# Autodesk Inventor assembly: KN-00-03-00
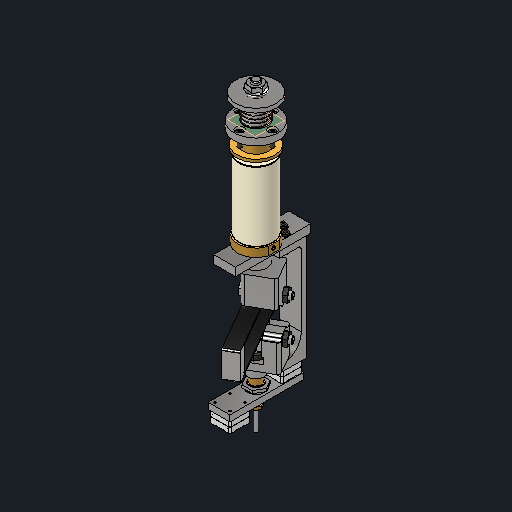
[picture p0: Inventor's stored thumbnail of the model, 512x512]
Saved by Autodesk Inventor 2025.2 (Build 292293000, 293)
## iProperties
Created: 2025-03-24
Part Number: KN-00-03-00
Document SubType Name: Assembly
Designer: Kacper Mik
Mass: 1101.42 g
Surface Area: 706.876 cm^2
Volume: 148.025 cm^3
Density: 7.44076 g/cm^3
Author: Kacper Mik
## Documents named in this file (32)
- C:\Users\kacpe\Documents\STUDIA\INŻYNIERKA\Nanotwardościomierz\Nanotwardosciomierz inventor\03-00-zesp_referencji.iam
- 03-00-zesp_wgłębnika.iam
- C:\Users\kacpe\Documents\STUDIA\INŻYNIERKA\Nanotwardościomierz\Nanotwardosciomierz inventor\Pobrane\Uchwyt do wgłębnika.ipt
- C:\Users\kacpe\Documents\STUDIA\INŻYNIERKA\Nanotwardościomierz\Nanotwardosciomierz inventor\02-01-ind_plytkaC1.ipt
- C:\Users\kacpe\Documents\STUDIA\INŻYNIERKA\Nanotwardościomierz\Nanotwardosciomierz inventor\02-01-ind_tulejaC1.ipt
- C:\Users\kacpe\Documents\STUDIA\INŻYNIERKA\Nanotwardościomierz\Nanotwardosciomierz inventor\02-01-dociskC1.ipt
- C:\Users\kacpe\Documents\STUDIA\INŻYNIERKA\Nanotwardościomierz\Nanotwardosciomierz inventor\02-04-ind_trzpien.ipt
- C:\Users\kacpe\Documents\STUDIA\INŻYNIERKA\Nanotwardościomierz\Nanotwardosciomierz inventor\P-025.40H Piezo Ring Actuators.ipt
- C:\Users\kacpe\Documents\STUDIA\INŻYNIERKA\Nanotwardościomierz\Nanotwardosciomierz inventor\Łożysko liniowe z kołnierzem okrągłym LMF08UU-L.ipt
- C:\Users\kacpe\Documents\STUDIA\INŻYNIERKA\Nanotwardościomierz\Nanotwardosciomierz inventor\02-06-tuleja_A0.ipt
- C:\Users\kacpe\Documents\STUDIA\INŻYNIERKA\Nanotwardościomierz\Nanotwardosciomierz inventor\CC\en-US\ISO 7045  H\ISO 7045 - M3 x 8_ - 4.8 - H - ISO.ipt
- C:\Users\kacpe\Documents\STUDIA\INŻYNIERKA\Nanotwardościomierz\Nanotwardosciomierz inventor\zesp_czujnikow.iam
- C:\Users\kacpe\Documents\STUDIA\INŻYNIERKA\Nanotwardościomierz\Nanotwardosciomierz inventor\02-07-zawieszka_K1\02-07-zawieszka_K1.ipt
- C:\Users\kacpe\Documents\STUDIA\INŻYNIERKA\Nanotwardościomierz\Nanotwardosciomierz inventor\CC\en-US\ISO 4036(2)\ISO 4036 - M6(2).ipt
- C:\Users\kacpe\Documents\STUDIA\INŻYNIERKA\Nanotwardościomierz\Nanotwardosciomierz inventor\CC\en-US\ISO 4036(2)\ISO 4036 - M5(2).ipt
- C:\Users\kacpe\Documents\STUDIA\INŻYNIERKA\Nanotwardościomierz\Nanotwardosciomierz inventor\Zawias.ipt
- C:\Users\kacpe\Documents\STUDIA\INŻYNIERKA\Nanotwardościomierz\Nanotwardosciomierz inventor\CC\en-US\ISO 4014(2)\ISO 4014 - M5 x 25 - ISO.ipt
- C:\Users\kacpe\Documents\STUDIA\INŻYNIERKA\Nanotwardościomierz\Nanotwardosciomierz inventor\02-08-ind_trzpien_gora.ipt
- C:\Users\kacpe\Documents\STUDIA\INŻYNIERKA\Nanotwardościomierz\Nanotwardosciomierz inventor\02-09-plyta_C1.ipt
- C:\Users\kacpe\Documents\STUDIA\INŻYNIERKA\Nanotwardościomierz\Nanotwardosciomierz inventor\02-11-plyta_dolnaA1.ipt
- C:\Users\kacpe\Documents\STUDIA\INŻYNIERKA\Nanotwardościomierz\Nanotwardosciomierz inventor\02-12-tuleja_dolnaA1.ipt
- C:\Users\kacpe\Documents\STUDIA\INŻYNIERKA\Nanotwardościomierz\Nanotwardosciomierz inventor\CC\en-US\ISO 7089\ISO 7089 - 2 - 140 HV(1).ipt
- C:\Users\kacpe\Documents\STUDIA\INŻYNIERKA\Nanotwardościomierz\Nanotwardosciomierz inventor\CC\en-US\ISO 7045  H\ISO 7045 - M2 x 14_ - 4.8 - H - ISO.ipt
- C:\Users\kacpe\Documents\STUDIA\INŻYNIERKA\Nanotwardościomierz\Nanotwardosciomierz inventor\CC\en-US\ISO 4036(2)\ISO 4036 - M2(2).ipt
- C:\Users\kacpe\Documents\STUDIA\INŻYNIERKA\Nanotwardościomierz\Nanotwardosciomierz inventor\CC\en-US\ISO 7045  H\ISO 7045 - M2 x 8_ - 4.8 - H - ISO.ipt
- C:\Users\kacpe\Documents\STUDIA\INŻYNIERKA\Nanotwardościomierz\Nanotwardosciomierz inventor\CC\en-US\ISO 4766(2)\ISO 4766 - M3 x 8 - ISO.ipt
- C:\Users\kacpe\Documents\STUDIA\INŻYNIERKA\Nanotwardościomierz\Nanotwardosciomierz inventor\02-14-podkladka_K3.ipt
- C:\Users\kacpe\Documents\STUDIA\INŻYNIERKA\Nanotwardościomierz\Nanotwardosciomierz inventor\CC\en-US\ISO 4161\ISO 4161 - M6(1).ipt
- C:\Users\kacpe\Documents\STUDIA\INŻYNIERKA\Nanotwardościomierz\Nanotwardosciomierz inventor\02-15-sprezyna_K3.ipt
- C:\Users\kacpe\Documents\STUDIA\INŻYNIERKA\Nanotwardościomierz\Nanotwardosciomierz inventor\02-15-prowadzenie_K3.ipt
- C:\Users\kacpe\Documents\STUDIA\INŻYNIERKA\Nanotwardościomierz\Nanotwardosciomierz inventor\03-01-glowica_referencyjna.ipt
- C:\Users\kacpe\Documents\STUDIA\INŻYNIERKA\Nanotwardościomierz\Nanotwardosciomierz inventor\CC\en-US\CNS 4355\CNS 4355 - M 1,4 x 6.ipt
## Components (59 placed, 30 different names)
1. 03-01-glowica_referencyjna:1
2. CNS 4355 M 1,4 x 6:5 — Insert:65
3. CNS 4355 M 1,4 x 6:6 — Insert:64
4. CNS 4355 M 1,4 x 6:7 — Insert:63
5. CNS 4355 M 1,4 x 6:8 — Insert:62
6. zesp_czujnikow:3 [sub-assembly] — Insert:66, Insert:67, Insert:68, Insert:69, Insert:70, Insert:71
7. CNS 4355 M 1,4 x 6:9 — Insert:71
8. CNS 4355 M 1,4 x 6:10 — Insert:70
9. CNS 4355 M 1,4 x 6:11 — Insert:69
10. CNS 4355 M 1,4 x 6:12 — Insert:68
11. 02-14-podkladka_K3:1 — Insert:45, Insert:46
12. 02-15-prowadzenie_K3:1 — Insert:55
13. 02-15-sprezyna_K3:1 — Mate:20, Mate:21
14. 02-01-ind_plytkaC1:1 — Angle:1, Insert:2, Insert:7, Insert:15, Insert:16, Insert:66, Insert:67
15. 02-02-ind_tulejaC1:1 — Insert:2, Insert:5, Insert:6
16. 02-03-docisk:1 — Insert:7, Angle:2
17. 02-04-ind_trzpien_dolny:1 — Insert:6, Insert:19
18. 02-06-tuleja_A0:1 — Insert:12, Insert:56
19. 02-07-zawieszka_K1:1 — Angle:4, Insert:21, Angle:5, Insert:22, Angle:6, Insert:24, Insert:25
20. 02-08-zawias — Insert:19, Insert:20, Insert:21, Angle:5, Insert:23
21. 02-08-zawias:2 — Angle:6, Insert:24, Insert:26, Insert:27, Insert:28
22. 02-09-plyta_C1:1 — Insert:29, Insert:30, Insert:32, Insert:51, Insert:52
23. 02-10-ind_trzpien_gora:1 — Insert:27, Insert:31, Insert:45
24. 02-11-plyta_dolnaA1:1 — Insert:31, Angle:7, Insert:36, Insert:40, Insert:53, Insert:54, Angle:8
25. 02-12-tuleja_dolnaA1:1 — Insert:40, Insert:41, Insert:42, Insert:43, Insert:44, Angle:8
26. CNS 4355 M 1,4 x 6:4 — Insert:59
27. CNS 4355 M 1,4 x 6:2 — Insert:60
28. CNS 4355 M 1,4 x 6:3 — Insert:58
29. CNS 4355 M 1,4 x 6:1 — Insert:61
30. ISO 7089 2:7 — Insert:53
31. ISO 7089 2:6 — Insert:52
32. ISO 4036 M2:3
33. ISO 7089 2:5 — Insert:54
34. ISO 7045 H M2 x 14 - 4.8 - H:3
35. ISO 4036 M2:2
36. ISO 7089 2:4 — Insert:51
37. ISO 7045 H M2 x 14 - 4.8 - H:2
38. ISO 4161 M6:1 — Insert:46
39. ISO 4766 M3 x 8:1 — Insert:43
40. ISO 7045 H M2 x 8 - 4.8 - H:2 — Insert:42
41. ISO 7045 H M2 x 8 - 4.8 - H:1 — Insert:41
42. ISO 7089 2:3 — Insert:36, Insert:37
43. ISO 4036 M2:1 — Insert:37
44. ISO 7089 2:1 — Insert:32, Insert:33
45. ISO 7045 H M2 x 14 - 4.8 - H:1 — Insert:33
46. ISO 4014 M5 x 25:2 — Insert:25
47. ISO 4036 M5:2 — Insert:26
48. ISO 4036 M6:2 — Insert:28
49. ISO 4036 M5:1 — Insert:23
50. ISO 4036 M6:1 — Insert:20
51. ISO 4014 M5 x 25:1 — Insert:22
52. ISO 7045 H M3 x 8 - 4.8 - H:4 — Mate:8
53. ISO 7045 H M3 x 8 - 4.8 - H:3 — Mate:6
54. ISO 7045 H M3 x 8 - 4.8 - H:2 — Mate:4
55. ISO 7045 H M3 x 8 - 4.8 - H:1 — Mate:2
56. P-025.40H Piezo Ring Actuators:1 — Insert:12, Insert:44
57. LMF08UU-L-Łożysko liniowe z kołnierzem okrągłym:1 — Angle:3, Mate:2, Mate:4, Mate:6, Mate:8, Mate:19, Mate:21, Insert:55, Insert:56
58. Uchwyt do wgłębnika:1 — Insert:5, Angle:2
59. zesp_czujnikow:2 [sub-assembly] — Insert:15, Insert:16, Insert:29, Insert:30, Insert:58, Insert:59, Insert:60, Insert:61, Insert:62, Insert:63, Insert:64, Insert:65
## Relationships (70: Insert 55, Angle 8, Mate 7)
- Angle:1 (0 deg): 02-01-ind_plytkaC1:1
- Insert:2: 02-01-ind_plytkaC1:1 ↔ 02-02-ind_tulejaC1:1
- Insert:5: 02-02-ind_tulejaC1:1 ↔ Uchwyt do wgłębnika:1
- Insert:6: 02-02-ind_tulejaC1:1 ↔ 02-04-ind_trzpien_dolny:1
- Insert:7: 02-01-ind_plytkaC1:1 ↔ 02-03-docisk:1
- Angle:2 (0 deg): 02-03-docisk:1 ↔ Uchwyt do wgłębnika:1
- Angle:3 (0 deg): LMF08UU-L-Łożysko liniowe z kołnierzem okrągłym:1
- Mate:2: ISO 7045 H M3 x 8 - 4.8 - H:1 ↔ LMF08UU-L-Łożysko liniowe z kołnierzem okrągłym:1
- Mate:4: ISO 7045 H M3 x 8 - 4.8 - H:2 ↔ LMF08UU-L-Łożysko liniowe z kołnierzem okrągłym:1
- Mate:6: ISO 7045 H M3 x 8 - 4.8 - H:3 ↔ LMF08UU-L-Łożysko liniowe z kołnierzem okrągłym:1
- Mate:8: ISO 7045 H M3 x 8 - 4.8 - H:4 ↔ LMF08UU-L-Łożysko liniowe z kołnierzem okrągłym:1
- Insert:12 (-0.2 mm): 02-06-tuleja_A0:1 ↔ P-025.40H Piezo Ring Actuators:1
- Insert:15: 02-01-ind_plytkaC1:1 ↔ zesp_czujnikow:2
- Insert:16: 02-01-ind_plytkaC1:1 ↔ zesp_czujnikow:2
- Angle:4 (60 deg): 02-07-zawieszka_K1:1
- Insert:19: 02-04-ind_trzpien_dolny:1 ↔ 02-08-zawias
- Insert:20: 02-08-zawias ↔ ISO 4036 M6:1
- Insert:21: 02-07-zawieszka_K1:1 ↔ 02-08-zawias
- Angle:5 (0 deg): 02-07-zawieszka_K1:1 ↔ 02-08-zawias
- Insert:22: 02-07-zawieszka_K1:1 ↔ ISO 4014 M5 x 25:1
- Insert:23: 02-08-zawias ↔ ISO 4036 M5:1
- Angle:6 (180 deg): 02-07-zawieszka_K1:1 ↔ 02-08-zawias:2
- Insert:24: 02-07-zawieszka_K1:1 ↔ 02-08-zawias:2
- Insert:25: 02-07-zawieszka_K1:1 ↔ ISO 4014 M5 x 25:2
- Insert:26: 02-08-zawias:2 ↔ ISO 4036 M5:2
- Insert:27: 02-08-zawias:2 ↔ 02-10-ind_trzpien_gora:1
- Insert:28: 02-08-zawias:2 ↔ ISO 4036 M6:2
- Insert:29: 02-09-plyta_C1:1 ↔ zesp_czujnikow:2
- Insert:30: 02-09-plyta_C1:1 ↔ zesp_czujnikow:2
- Insert:31: 02-10-ind_trzpien_gora:1 ↔ 02-11-plyta_dolnaA1:1
- Angle:7 (0 deg): 02-11-plyta_dolnaA1:1
- Insert:32: 02-09-plyta_C1:1 ↔ ISO 7089 2:1
- Insert:33: ISO 7089 2:1 ↔ ISO 7045 H M2 x 14 - 4.8 - H:1
- Insert:36: 02-11-plyta_dolnaA1:1 ↔ ISO 7089 2:3
- Insert:37: ISO 7089 2:3 ↔ ISO 4036 M2:1
- Mate:19: LMF08UU-L-Łożysko liniowe z kołnierzem okrągłym:1
- Insert:40: 02-11-plyta_dolnaA1:1 ↔ 02-12-tuleja_dolnaA1:1
- Insert:41: 02-12-tuleja_dolnaA1:1 ↔ ISO 7045 H M2 x 8 - 4.8 - H:1
- Insert:42: 02-12-tuleja_dolnaA1:1 ↔ ISO 7045 H M2 x 8 - 4.8 - H:2
- Insert:43 (0.35 mm): 02-12-tuleja_dolnaA1:1 ↔ ISO 4766 M3 x 8:1
- Insert:44: 02-12-tuleja_dolnaA1:1 ↔ P-025.40H Piezo Ring Actuators:1
- Insert:45: 02-14-podkladka_K3:1 ↔ 02-10-ind_trzpien_gora:1
- Insert:46: 02-14-podkladka_K3:1 ↔ ISO 4161 M6:1
- [Insert]: ISO 7089 2:4 ↔ ISO 7045 H M2 x 14 - 4.8 - H:2
- [Insert]: ISO 7089 2:5 ↔ ISO 4036 M2:2
- [Insert]: ISO 7089 2:6 ↔ ISO 7045 H M2 x 14 - 4.8 - H:3
- [Insert]: ISO 7089 2:7 ↔ ISO 4036 M2:3
- Insert:51: 02-09-plyta_C1:1 ↔ ISO 7089 2:4
- Insert:52: 02-09-plyta_C1:1 ↔ ISO 7089 2:6
- Insert:53: 02-11-plyta_dolnaA1:1 ↔ ISO 7089 2:7
- Insert:54: 02-11-plyta_dolnaA1:1 ↔ ISO 7089 2:5
- Mate:20: 02-15-sprezyna_K3:1
- Mate:21: 02-15-sprezyna_K3:1 ↔ LMF08UU-L-Łożysko liniowe z kołnierzem okrągłym:1
- Insert:55: 02-15-prowadzenie_K3:1 ↔ LMF08UU-L-Łożysko liniowe z kołnierzem okrągłym:1
- Insert:56 (1 mm): 02-06-tuleja_A0:1 ↔ LMF08UU-L-Łożysko liniowe z kołnierzem okrągłym:1
- Insert:58: CNS 4355 M 1,4 x 6:3 ↔ zesp_czujnikow:2
- Insert:59: CNS 4355 M 1,4 x 6:4 ↔ zesp_czujnikow:2
- Insert:60: CNS 4355 M 1,4 x 6:2 ↔ zesp_czujnikow:2
- Insert:61: CNS 4355 M 1,4 x 6:1 ↔ zesp_czujnikow:2
- Insert:62: CNS 4355 M 1,4 x 6:8 ↔ zesp_czujnikow:2
- Insert:63: CNS 4355 M 1,4 x 6:7 ↔ zesp_czujnikow:2
- Insert:64: CNS 4355 M 1,4 x 6:6 ↔ zesp_czujnikow:2
- Insert:65: CNS 4355 M 1,4 x 6:5 ↔ zesp_czujnikow:2
- Insert:66: zesp_czujnikow:3 ↔ 02-01-ind_plytkaC1:1
- Insert:67: zesp_czujnikow:3 ↔ 02-01-ind_plytkaC1:1
- Insert:68: zesp_czujnikow:3 ↔ CNS 4355 M 1,4 x 6:12
- Insert:69: zesp_czujnikow:3 ↔ CNS 4355 M 1,4 x 6:11
- Insert:70: zesp_czujnikow:3 ↔ CNS 4355 M 1,4 x 6:10
- Insert:71: zesp_czujnikow:3 ↔ CNS 4355 M 1,4 x 6:9
- Angle:8 (0 deg): 02-11-plyta_dolnaA1:1 ↔ 02-12-tuleja_dolnaA1:1
## Named parameters: d83_d66 = 0 mm, d84_d70 = 0 mm, d85_d66 = 0 mm, d86_d70 = 0 mm
